# Autodesk Inventor assembly: Assembly2
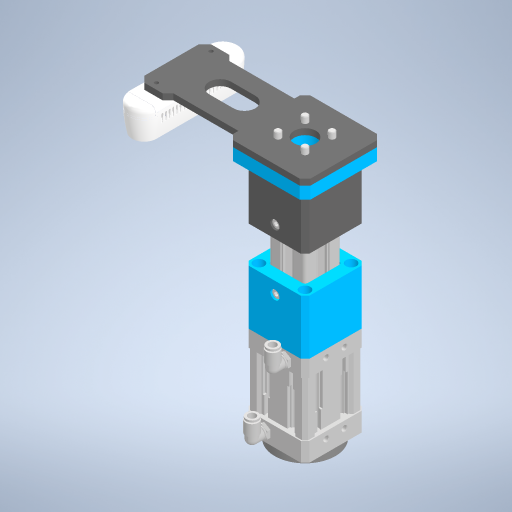
[picture p0: Inventor's stored thumbnail of the model, 512x512]
Saved by Autodesk Inventor 2023 (Build 270158000, 158)
## iProperties
Created: 2022-05-24
Part Number: Assembly2
Document SubType Name: Assembly
Designer: romanp
Author: romanp
## Documents named in this file (14)
- C:\Users\romanp\Downloads\SMC_EE_MHM-32D1-X6400\Assembly_SMC_EE.iam
- C:\Users\romanp\Downloads\SMC_EE_MHM-32D1-X6400\MHM-32D1-X6400(0).iam
- C:\Users\romanp\Downloads\SMC_EE_MHM-32D1-X6400\Part_Top_a_Blue.ipt
- C:\Users\romanp\Downloads\SMC_EE_MHM-32D1-X6400\Part_Bottom_Blue.ipt
- C:\Users\romanp\Downloads\SMC_EE_MHM-32D1-X6400\Part_Middle_Black.ipt
- C:\Users\romanp\Downloads\SMC_EE_MHM-32D1-X6400\ITEM30x30x100.ipt
- C:\Users\romanp\Downloads\SMC_EE_MHM-32D1-X6400\M5x25.ipt
- C:\Users\romanp\Downloads\SMC_EE_MHM-32D1-X6400\M4_nut.ipt
- C:\Users\romanp\Downloads\SMC_EE_MHM-32D1-X6400\Part_Type_1_Black.ipt
- C:\Users\romanp\Downloads\SMC_EE_MHM-32D1-X6400\IntelRealsense_D435.ipt
- C:\Users\romanp\Downloads\SMC_EE_MHM-32D1-X6400\M4x10.ipt
- C:\Users\romanp\Downloads\SMC_EE_MHM-32D1-X6400\M5x20.ipt
- C:\Users\romanp\Downloads\SMC_EE_MHM-32D1-X6400\M4x20.ipt
- C:\Users\romanp\Downloads\SMC_EE_MHM-32D1-X6400\KQ2L06-01N.ipt
## Components (29 placed, 14 different names)
1. Part_Top_a_Blue — Insert:15, Insert:16, Insert:25, Insert:45, Insert:46, Insert:47, Insert:54
2. M5x25:1
3. Part_Type_1_Black — Insert:15, Insert:16, Insert:17, Insert:18
4. IntelRealsense_D435:1 — Insert:17, Insert:18
5. M4x10:5
6. M4x20:1
7. M4_nut:3 — Insert:25
8. M4x10:7
9. ITEM30x30x100:3
10. MHM-32D1-X6400(0):3 [sub-assembly] — Insert:51, Insert:52, Insert:53
11. M5x75:2
12. M4x10:8
13. M4x10:9
14. M5x75:3
15. M5x75:4
16. M5x75:5
17. M5x25:2
18. M5x25:3
19. M5x25:4
20. M4_nut:4 — Insert:46
21. M4_nu:5 — Insert:47
22. M4_nu:6 — Insert:45
23. M4x20:5
24. M4x20:6
25. M4x20:7
26. KQ2L06-01N:3 — Insert:51
27. KQ2L06-01N:4 — Insert:52
28. Part_Middle_Black:1 — Insert:54
29. Part_Bottom_Blue:1 — Insert:53
## Relationships (12: Insert 12)
- Insert:15: Part_Top_a_Blue ↔ Part_Type_1_Black
- Insert:16: Part_Top_a_Blue ↔ Part_Type_1_Black
- Insert:17: Part_Type_1_Black ↔ IntelRealsense_D435:1
- Insert:18: Part_Type_1_Black ↔ IntelRealsense_D435:1
- Insert:25: Part_Top_a_Blue ↔ M4_nut:3
- Insert:45: Part_Top_a_Blue ↔ M4_nu:6
- Insert:46: Part_Top_a_Blue ↔ M4_nut:4
- Insert:47: Part_Top_a_Blue ↔ M4_nu:5
- Insert:51: MHM-32D1-X6400(0):3 ↔ KQ2L06-01N:3
- Insert:52: MHM-32D1-X6400(0):3 ↔ KQ2L06-01N:4
- Insert:53: MHM-32D1-X6400(0):3 ↔ Part_Bottom_Blue:1
- Insert:54: Part_Top_a_Blue ↔ Part_Middle_Black:1
